# Autodesk Inventor assembly: Elesembly
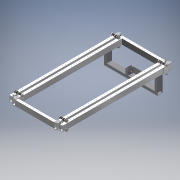
[picture p0: Inventor's stored thumbnail of the model, 180x180]
Saved by Autodesk Inventor 2018 (Build 220112000, 112)
## iProperties
Created: 2018-08-29
Part Number: Elesembly
Document SubType Name: Assembly
Designer: baoan
Author: baoan
## Documents named in this file (9)
- C:\Users\baoan\Documents\Inventor\Elevator\Elesembly.iam
- C:\Users\baoan\Documents\Inventor\Elevator\elevator_12''_frame.ipt
- C:\Users\baoan\Documents\Inventor\Elevator\front_bearings.iam
- C:\Users\baoan\Documents\Inventor\Elevator\Side_bearings.iam
- C:\Users\baoan\Documents\Inventor\Elevator\Horizontal_frame_2nd_stage.ipt
- C:\Users\baoan\Documents\Inventor\Elevator\Elevator_stationary_extender.ipt
- C:\Users\baoan\Documents\Inventor\Elevator\Stationary_Horizontal_extender.ipt
- C:\Users\baoan\Documents\Inventor\Elevator\Extender_pulley_gusset.ipt
- C:\Users\baoan\Documents\Inventor\Elevator\Pulley_holder.ipt
## Components (20 placed, 8 different names)
1. elevator_12''_frame:1 — Flush:5, Mate:5, Flush:8, Flush:9, Flush:10, Tangent:1, Tangent:2, Tangent:3, Tangent:5, Tangent:7, Mate:11, Flush:16, Flush:17, Mate:12, Flush:18, Mate:15, Flush:25, Flush:26
2. elevator_12''_frame:2 — Flush:6, Mate:5, Flush:8, Flush:9, Angle:1, Tangent:4, Mate:9, Flush:13, Mate:10, Flush:14, Flush:15, Tangent:9, Mate:16, Flush:27, Flush:28
3. elevator_12''_frame:3 — Mate:2, Flush:3, Flush:4, Flush:6, Flush:7, Angle:1, Mate:8, Flush:12, Tangent:6, Tangent:8, Flush:21, Flush:22
4. elevator_12''_frame:4 — Mate:1, Flush:1, Flush:2, Flush:5, Flush:7, Flush:10, Mate:6, Mate:7, Flush:11, Tangent:10, Tangent:11, Tangent:12, Mate:13, Flush:19, Flush:20, Mate:14, Flush:23, Flush:24
5. front_bearings:1 [sub-assembly] — Mate:2, Flush:3, Flush:4, Tangent:9
6. front_bearings:2 [sub-assembly] — Mate:1, Flush:1, Flush:2, Tangent:1
7. Side_bearings:1 [sub-assembly] — Mate:6, Mate:7, Tangent:2, Tangent:3, Flush:11, Tangent:5, Tangent:7
8. Side_bearings:2 [sub-assembly] — Mate:8, Tangent:4, Flush:12
9. front_bearings:3 [sub-assembly] — Mate:10, Flush:14, Flush:15, Tangent:8
10. Side_bearings:3 [sub-assembly] — Mate:9, Tangent:6, Flush:13
11. Side_bearings:4 [sub-assembly] — Mate:12, Tangent:11, Tangent:12, Flush:18
12. front_bearings:4 [sub-assembly] — Mate:11, Flush:16, Flush:17, Tangent:10
13. Horizontal_frame_2nd_stage:1 — Mate:13, Flush:19, Flush:20, Flush:21, Flush:22
14. Horizontal_frame_2nd_stage:2 — Mate:14, Flush:23, Flush:24
15. Elevator_stationary_extender:1 — Mate:15, Flush:25, Flush:26, Flush:29, Flush:30
16. Elevator_stationary_extender:2 — Mate:16, Flush:27, Flush:28, Mate:17
17. Stationary_Horizontal_extender:1 — Mate:17, Flush:29, Flush:30, Mate:18, Flush:31
18. Extender_pulley_gusset:1 — Mate:18, Flush:31, Mate:19, Flush:32, Flush:33, Mate:20, Flush:34, Flush:35
19. Pulley_holder:1 — Mate:19, Flush:32, Flush:33
20. Pulley_holder:2 — Mate:20, Flush:34, Flush:35
## Relationships (66: Flush 35, Mate 18, Tangent 12, Angle 1)
- Mate:1: elevator_12''_frame:4 ↔ front_bearings:2
- Flush:1: elevator_12''_frame:4 ↔ front_bearings:2
- Flush:2: elevator_12''_frame:4 ↔ front_bearings:2
- Mate:2: elevator_12''_frame:3 ↔ front_bearings:1
- Flush:3: elevator_12''_frame:3 ↔ front_bearings:1
- Flush:4: elevator_12''_frame:3 ↔ front_bearings:1
- Flush:5: elevator_12''_frame:1 ↔ elevator_12''_frame:4
- Flush:6: elevator_12''_frame:2 ↔ elevator_12''_frame:3
- Flush:7: elevator_12''_frame:3 ↔ elevator_12''_frame:4
- Mate:5 (-508 mm): elevator_12''_frame:1 ↔ elevator_12''_frame:2
- Flush:8: elevator_12''_frame:1 ↔ elevator_12''_frame:2
- Flush:9: elevator_12''_frame:1 ↔ elevator_12''_frame:2
- Flush:10: elevator_12''_frame:1 ↔ elevator_12''_frame:4
- Angle:1 (180 deg): elevator_12''_frame:2 ↔ elevator_12''_frame:3
- Mate:6: elevator_12''_frame:4 ↔ Side_bearings:1
- Mate:7: elevator_12''_frame:4 ↔ Side_bearings:1
- Tangent:1: elevator_12''_frame:1 ↔ front_bearings:2
- Tangent:2: elevator_12''_frame:1 ↔ Side_bearings:1
- Tangent:3: elevator_12''_frame:1 ↔ Side_bearings:1
- Flush:11 (40.64 mm): elevator_12''_frame:4 ↔ Side_bearings:1
- Mate:8: elevator_12''_frame:3 ↔ Side_bearings:2
- Tangent:4: elevator_12''_frame:2 ↔ Side_bearings:2
- Tangent:5: elevator_12''_frame:1 ↔ Side_bearings:1
- Flush:12 (40.64 mm): elevator_12''_frame:3 ↔ Side_bearings:2
- Mate:9: elevator_12''_frame:2 ↔ Side_bearings:3
- Tangent:6: elevator_12''_frame:3 ↔ Side_bearings:3
- Tangent:7: elevator_12''_frame:1 ↔ Side_bearings:1
- Flush:13 (40.64 mm): elevator_12''_frame:2 ↔ Side_bearings:3
- Mate:10: elevator_12''_frame:2 ↔ front_bearings:3
- Flush:14: elevator_12''_frame:2 ↔ front_bearings:3
- Flush:15: elevator_12''_frame:2 ↔ front_bearings:3
- Tangent:8: elevator_12''_frame:3 ↔ front_bearings:3
- Tangent:9: elevator_12''_frame:2 ↔ front_bearings:1
- Mate:11: elevator_12''_frame:1 ↔ front_bearings:4
- Flush:16: elevator_12''_frame:1 ↔ front_bearings:4
- Flush:17: elevator_12''_frame:1 ↔ front_bearings:4
- Tangent:10: elevator_12''_frame:4 ↔ front_bearings:4
- Mate:12: elevator_12''_frame:1 ↔ Side_bearings:4
- Tangent:11: elevator_12''_frame:4 ↔ Side_bearings:4
- Tangent:12: elevator_12''_frame:4 ↔ Side_bearings:4
- Flush:18 (40.64 mm): elevator_12''_frame:1 ↔ Side_bearings:4
- Mate:13: elevator_12''_frame:4 ↔ Horizontal_frame_2nd_stage:1
- Flush:19: elevator_12''_frame:4 ↔ Horizontal_frame_2nd_stage:1
- Flush:20: elevator_12''_frame:4 ↔ Horizontal_frame_2nd_stage:1
- Flush:21: elevator_12''_frame:3 ↔ Horizontal_frame_2nd_stage:1
- Flush:22: elevator_12''_frame:3 ↔ Horizontal_frame_2nd_stage:1
- Mate:14: elevator_12''_frame:4 ↔ Horizontal_frame_2nd_stage:2
- Flush:23: elevator_12''_frame:4 ↔ Horizontal_frame_2nd_stage:2
- Flush:24: elevator_12''_frame:4 ↔ Horizontal_frame_2nd_stage:2
- Mate:15: elevator_12''_frame:1 ↔ Elevator_stationary_extender:1
- Flush:25: elevator_12''_frame:1 ↔ Elevator_stationary_extender:1
- Flush:26 (88.9 mm): elevator_12''_frame:1 ↔ Elevator_stationary_extender:1
- Mate:16: elevator_12''_frame:2 ↔ Elevator_stationary_extender:2
- Flush:27 (88.9 mm): elevator_12''_frame:2 ↔ Elevator_stationary_extender:2
- Flush:28: elevator_12''_frame:2 ↔ Elevator_stationary_extender:2
- Mate:17: Elevator_stationary_extender:2 ↔ Stationary_Horizontal_extender:1
- Flush:29: Elevator_stationary_extender:1 ↔ Stationary_Horizontal_extender:1
- Flush:30: Elevator_stationary_extender:1 ↔ Stationary_Horizontal_extender:1
- Mate:18: Stationary_Horizontal_extender:1 ↔ Extender_pulley_gusset:1
- Flush:31: Stationary_Horizontal_extender:1 ↔ Extender_pulley_gusset:1
- Mate:19: Extender_pulley_gusset:1 ↔ Pulley_holder:1
- Flush:32: Extender_pulley_gusset:1 ↔ Pulley_holder:1
- Flush:33: Extender_pulley_gusset:1 ↔ Pulley_holder:1
- Mate:20: Extender_pulley_gusset:1 ↔ Pulley_holder:2
- Flush:34: Extender_pulley_gusset:1 ↔ Pulley_holder:2
- Flush:35: Extender_pulley_gusset:1 ↔ Pulley_holder:2
